# Autodesk Inventor assembly: wheel mount
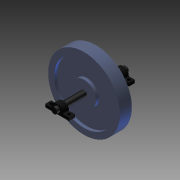
[picture p0: Inventor's stored thumbnail of the model, 180x180]
Saved by Autodesk Inventor 2011 (Build 150239000, 239)
## iProperties
Created: 2013-01-19
Part Number: wheel mount
Document SubType Name: Assembly
Designer: Christopher
Author: Christopher
## Documents named in this file (4)
- F:\Users\Christopher\Documents\GitHub\2013CAD\2013 robot\forklift\Pneumatics and frame grabbers\wheel mount.iam
- F:\Users\Christopher\Documents\GitHub\2013CAD\2013 robot\forklift\Misc parts\.5inch_side_bearing.ipt
- F:\Users\Christopher\Documents\GitHub\2013CAD\2013 robot\forklift\robot parts\example_wheel_6inch_.5axle.ipt
- F:\Users\Christopher\Documents\GitHub\2013CAD\2013 robot\forklift\robot parts\wheelaxle.ipt
## Components (4 placed, 3 different names)
1. .5inch_side_bearing:1 — Insert:2, Flush:1
2. .5inch_side_bearing:2 — Insert:1, Flush:1
3. example_wheel_6inch_.5axle:1 — Insert:3
4. wheelaxle:1 — Insert:1, Insert:2, Insert:3
## Relationships (4: Insert 3, Flush 1)
- Insert:1 (-6.35 mm): .5inch_side_bearing:2 ↔ wheelaxle:1
- Insert:2 (6.35 mm): .5inch_side_bearing:1 ↔ wheelaxle:1
- Flush:1: .5inch_side_bearing:1 ↔ .5inch_side_bearing:2
- Insert:3 (63.5 mm): example_wheel_6inch_.5axle:1 ↔ wheelaxle:1
